# Autodesk Inventor assembly: Shooter P1
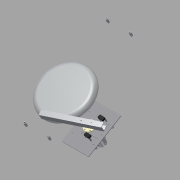
[picture p0: Inventor's stored thumbnail of the model, 180x180]
Saved by Autodesk Inventor 2013 (Build 170138000, 138)
## iProperties
Created: 2013-02-08
Part Number: Shooter P1
Document SubType Name: Assembly
Designer: Naphat
Author: Naphat
## Documents named in this file (11)
- C:\Autodesk\gruntmaster6000-cad\Prototypes\Shooter Firing Pin\Shooter P1.iam
- C:\Autodesk\gruntmaster6000-cad\Prototypes\Shooter Firing Pin\Mounting Plate.ipt
- C:\Autodesk\gruntmaster6000-cad\Imported Components\Motors\PG27\PG27.ipt
- C:\Autodesk\gruntmaster6000-cad\Imported Components\Motors\8mm-key-hub\8mm-key-hub.ipt
- C:\Autodesk\gruntmaster6000-cad\Imported Components\Motors\4x4x12 PG-27 Machine Key.ipt
- C:\Autodesk\gruntmaster6000-cad\Frisbee.ipt
- C:\Autodesk\gruntmaster6000-cad\Imported Components\Microswitch\SEN_Microswitch_V7-2B17D8-048.ipt
- C:\Autodesk\gruntmaster6000-cad\Prototypes\Shooter Firing Pin\.25in x 1 in Spacer.ipt
- C:\Autodesk\gruntmaster6000-cad\Prototypes\Shooter Firing Pin\Microswitch Spacer.ipt
- C:\Autodesk\gruntmaster6000-cad\Rack\Rack - Back.ipt
- C:\Autodesk\gruntmaster6000-cad\Prototypes\Shooter Firing Pin\Firing Arm.ipt
## Components (24 placed, 10 different names)
1. Frisbee:1
2. Mounting Plate:1 — Mate:3, Mate:17, Mate:18, Mate:19, Mate:20, Mate:21, Mate:22, Mate:23, Mate:24, Mate:25, Mate:26, Mate:27, Mate:28, Mate:29, Flush:5, Flush:6, Mate:50, Mate:56
3. PG27:1 — Mate:3, Mate:5, Mate:6, Flush:2, Mate:7, Mate:8, Mate:17
4. 8mm-key-hub:1 — Mate:7, Mate:8, Mate:63, Mate:64, Mate:65
5. 4x4x12 PG-27 Machine Key:1 — Mate:5, Mate:6, Flush:2
6. Firing Arm:1 — Mate:63, Mate:64, Mate:65
7. SEN_Microswitch_V7-2B17D8-048:1 — Flush:4, Mate:47, Flush:7, Mate:53, Mate:54, Mate:55
8. SEN_Microswitch_V7-2B17D8-048:2 — Flush:4, Flush:5, Flush:6, Mate:47, Flush:7, Mate:48, Mate:49, Mate:51, Mate:52
9. .25in x 1 in Spacer:1 — Mate:22, Mate:27
10. .25in x 1 in Spacer:2 — Mate:23, Mate:28
11. .25in x 1 in Spacer:3 — Mate:18, Mate:19
12. .25in x 1 in Spacer:4 — Mate:21, Mate:26
13. .25in x 1 in Spacer:5 — Mate:20, Mate:25
14. .25in x 1 in Spacer:6 — Mate:24, Mate:29
15. .25in x 1 in Spacer:7
16. .25in x 1 in Spacer:8
17. .25in x 1 in Spacer:9
18. .25in x 1 in Spacer:10
19. Microswitch Spacer:1 — Mate:51, Mate:52
20. Microswitch Spacer:2 — Mate:48, Mate:49, Mate:50
21. Microswitch Spacer:3 — Mate:53, Mate:54
22. Microswitch Spacer:4 — Mate:55, Mate:56
23. Rack - Back:1 — Mate:58
24. Rack - Back:2 — Mate:58
## Relationships (37: Mate 32, Flush 5)
- Mate:3: Mounting Plate:1 ↔ PG27:1
- Mate:5: PG27:1 ↔ 4x4x12 PG-27 Machine Key:1
- Mate:6: PG27:1 ↔ 4x4x12 PG-27 Machine Key:1
- Flush:2 (-4 mm): PG27:1 ↔ 4x4x12 PG-27 Machine Key:1
- Mate:7: PG27:1 ↔ 8mm-key-hub:1
- Mate:8: PG27:1 ↔ 8mm-key-hub:1
- Flush:4: SEN_Microswitch_V7-2B17D8-048:1 ↔ SEN_Microswitch_V7-2B17D8-048:2
- Mate:17: Mounting Plate:1 ↔ PG27:1
- Mate:18: Mounting Plate:1 ↔ .25in x 1 in Spacer:3
- Mate:19: Mounting Plate:1 ↔ .25in x 1 in Spacer:3
- Mate:20: Mounting Plate:1 ↔ .25in x 1 in Spacer:5
- Mate:21: Mounting Plate:1 ↔ .25in x 1 in Spacer:4
- Mate:22: Mounting Plate:1 ↔ .25in x 1 in Spacer:1
- Mate:23: Mounting Plate:1 ↔ .25in x 1 in Spacer:2
- Mate:24: Mounting Plate:1 ↔ .25in x 1 in Spacer:6
- Mate:25: Mounting Plate:1 ↔ .25in x 1 in Spacer:5
- Mate:26: Mounting Plate:1 ↔ .25in x 1 in Spacer:4
- Mate:27: Mounting Plate:1 ↔ .25in x 1 in Spacer:1
- Mate:28: Mounting Plate:1 ↔ .25in x 1 in Spacer:2
- Mate:29: Mounting Plate:1 ↔ .25in x 1 in Spacer:6
- Flush:5 (35.2552 mm): Mounting Plate:1 ↔ SEN_Microswitch_V7-2B17D8-048:2
- Flush:6 (59.2836 mm): Mounting Plate:1 ↔ SEN_Microswitch_V7-2B17D8-048:2
- Mate:47 (70.4596 mm): SEN_Microswitch_V7-2B17D8-048:1 ↔ SEN_Microswitch_V7-2B17D8-048:2
- Flush:7: SEN_Microswitch_V7-2B17D8-048:1 ↔ SEN_Microswitch_V7-2B17D8-048:2
- Mate:48: SEN_Microswitch_V7-2B17D8-048:2 ↔ Microswitch Spacer:2
- Mate:49: SEN_Microswitch_V7-2B17D8-048:2 ↔ Microswitch Spacer:2
- Mate:50: Mounting Plate:1 ↔ Microswitch Spacer:2
- Mate:51: SEN_Microswitch_V7-2B17D8-048:2 ↔ Microswitch Spacer:1
- Mate:52: SEN_Microswitch_V7-2B17D8-048:2 ↔ Microswitch Spacer:1
- Mate:53: SEN_Microswitch_V7-2B17D8-048:1 ↔ Microswitch Spacer:3
- Mate:54: SEN_Microswitch_V7-2B17D8-048:1 ↔ Microswitch Spacer:3
- Mate:55: SEN_Microswitch_V7-2B17D8-048:1 ↔ Microswitch Spacer:4
- Mate:56: Mounting Plate:1 ↔ Microswitch Spacer:4
- Mate:58: Rack - Back:1 ↔ Rack - Back:2
- Mate:63: 8mm-key-hub:1 ↔ Firing Arm:1
- Mate:64: 8mm-key-hub:1 ↔ Firing Arm:1
- Mate:65: 8mm-key-hub:1 ↔ Firing Arm:1
